# Autodesk Inventor assembly: var1
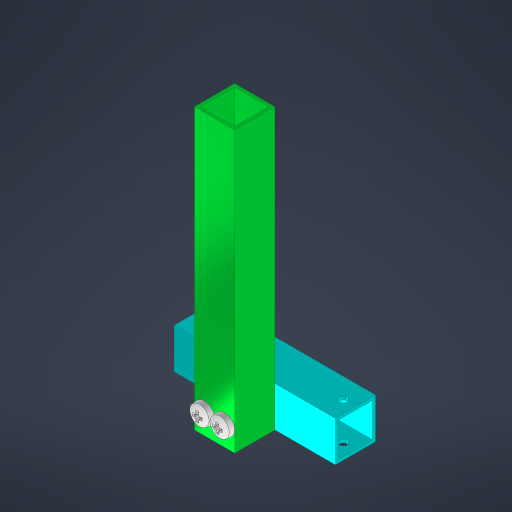
[picture p0: Inventor's stored thumbnail of the model, 512x512]
Saved by Autodesk Inventor 2024 (Build 280153000, 153)
## iProperties
Created: 2023-04-17
Part Number: var1
Document SubType Name: Assembly
Designer: user
Mass: 83.8365 g
Surface Area: 350.923 cm^2
Volume: 26.4237 cm^3
Density: 3.17278 g/cm^3
Author: user
## Documents named in this file (11)
- D:\Docs\Robot\3d\tests\var1\var1.iam
- D:\Docs\Robot\3d\tests\var1\1.ipt
- C:\Users\user\Documents\Inventor\Content Center Files\R2024\ru-RU\DIN 7985 (H)\DIN 7985 (H) - M5x45-H.ipt
- D:\Docs\Robot\3d\tests\var1\2.ipt
- C:\Users\user\Documents\Inventor\Content Center Files\R2024\ru-RU\DIN 985\DIN 985 - M5.ipt
- D:\Docs\Robot\3d\tests\var1\var1\AIP\FEA\eb2ulpa4g.fins
- D:\Docs\Robot\3d\tests\var1\var1\AIP\FEA\eb2ulpa4g.fsat
- D:\Docs\Robot\3d\tests\var1\var1\AIP\FEA\eb2ulpa4g.ftes
- D:\Docs\Robot\3d\tests\var1\var1\AIP\FEA\eb2ulpa4g.fwiz
- D:\Docs\Robot\3d\tests\var1\var1\AIP\FEA\eb2ulpa68.fmsh
- D:\Docs\Robot\3d\tests\var1\var1\AIP\FEA\eb2ulpa69.fres
## Components (6 placed, 4 different names)
1. 1:1 — Вставка:1, Вставка:2, Заподлицо:1
2. DIN 7985 (H) M5x45-H:1 — Вставка:1
3. DIN 7985 (H) M5x45-H:2 — Вставка:2
4. 2:1 — Заподлицо:1, Вставка:3, Вставка:4
5. DIN 985 - заменено на DIN EN ISO 10511 M5:1 — Вставка:3
6. DIN 985 - заменено на DIN EN ISO 10511 M5:2 — Вставка:4
## Relationships (5: Insert 4, Flush 1)
- Вставка:1 [Insert]: 1:1 ↔ DIN 7985 (H) M5x45-H:1
- Вставка:2 [Insert]: 1:1 ↔ DIN 7985 (H) M5x45-H:2
- Заподлицо:1 [Flush]: 1:1 ↔ 2:1
- Вставка:3 [Insert]: 2:1 ↔ DIN 985 - заменено на DIN EN ISO 10511 M5:1
- Вставка:4 [Insert]: 2:1 ↔ DIN 985 - заменено на DIN EN ISO 10511 M5:2
## Named parameters: sa_0 = 5000, sa_1 = 50000, sa_2 = 50000
note: some values were not read from the file. Shown as the stored number, unit unknown: "sa_0", "sa_1", "sa_2".
